# Autodesk Inventor assembly: test-model-2025dcm
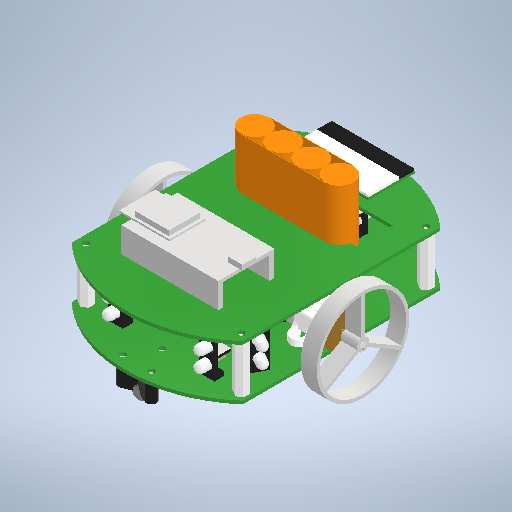
[picture p0: Inventor's stored thumbnail of the model, 512x512]
Saved by Autodesk Inventor 2025.3 (Build 293356000, 356)
## iProperties
Created: 2025-05-29
Part Number: test-model-2025dcm
Document SubType Name: Assembly
Designer: yamashita1
Author: yamashita1
## Documents named in this file (11)
- G:\マイドライブ\project\micro-mouse\3D-Model\test-model-2025dcm.iam
- G:\マイドライブ\project\micro-mouse\3D-Model\BaseBoard2.ipt
- G:\マイドライブ\project\micro-mouse\3D-Model\N20withBracket.iam
- G:\マイドライブ\project\micro-mouse\3D-Model\BallCaster-H16.ipt
- G:\マイドライブ\project\micro-mouse\3D-Model\D-Shaft_Wheel2.ipt
- G:\マイドライブ\project\micro-mouse\3D-Model\Photo-Sensor.iam
- G:\マイドライブ\project\micro-mouse\3D-Model\Spacer-M3H24.ipt
- G:\マイドライブ\project\micro-mouse\3D-Model\ESP32-DevKitC.ipt
- G:\マイドライブ\project\micro-mouse\3D-Model\NiMH-Battery.ipt
- G:\マイドライブ\project\micro-mouse\3D-Model\BaseBoard2B.ipt
- G:\マイドライブ\project\micro-mouse\3D-Model\AQM1602Y.ipt
## Components (19 placed, 10 different names)
1. BaseBoard2:1 — メイト:7, メイト:8, メイト:9, メイト:10, メイト:11, メイト:12, メイト:13, メイト:14, メイト:15, メイト:18, メイト:19, メイト:20, メイト:21, メイト:22, メイト:23, メイト:24, メイト:25, メイト:26, メイト:27, メイト:28, メイト:29, メイト:30, メイト:36
2. N20withBracket:1 [sub-assembly] — メイト:13, メイト:14, メイト:15, メイト:17, フラッシュ:2
3. N20withBracket:2 [sub-assembly] — メイト:10, メイト:11, メイト:12, メイト:16, フラッシュ:1
4. BallCaster-H16:1 — メイト:7, メイト:8, メイト:9
5. D-Shaft_Wheel2:1 — メイト:16, フラッシュ:1
6. D-Shaft_Wheel2:2 — メイト:17, フラッシュ:2
7. Photo-Sensor:1 [sub-assembly] — メイト:18
8. Photo-Sensor:2 [sub-assembly] — メイト:19
9. Photo-Sensor:3 [sub-assembly] — メイト:20
10. Photo-Sensor:4 [sub-assembly] — メイト:21
11. Photo-Sensor:5 [sub-assembly] — メイト:22
12. Spacer-M3H24:1 — メイト:23, メイト:29
13. Spacer-M3H24:2 — メイト:24, メイト:30, メイト:31, メイト:32
14. Spacer-M3H24:3 — メイト:25, メイト:27, メイト:33
15. Spacer-M3H24:4 — メイト:26, メイト:28
16. ESP32-DevKitC:1 — メイト:35
17. BaseBoard2B:1 — メイト:31, メイト:32, メイト:33, メイト:35
18. NiMH-Battery:1 — メイト:36
19. AQM1602Y:1
## Relationships (31: Mate 29, Flush 2)
- メイト:7 [Mate]: BaseBoard2:1 ↔ BallCaster-H16:1
- メイト:8 [Mate]: BaseBoard2:1 ↔ BallCaster-H16:1
- メイト:9 [Mate]: BaseBoard2:1 ↔ BallCaster-H16:1
- メイト:10 [Mate]: BaseBoard2:1 ↔ N20withBracket:2
- メイト:11 [Mate]: BaseBoard2:1 ↔ N20withBracket:2
- メイト:12 [Mate]: BaseBoard2:1 ↔ N20withBracket:2
- メイト:13 [Mate]: BaseBoard2:1 ↔ N20withBracket:1
- メイト:14 [Mate]: BaseBoard2:1 ↔ N20withBracket:1
- メイト:15 [Mate]: BaseBoard2:1 ↔ N20withBracket:1
- メイト:16 [Mate]: N20withBracket:2 ↔ D-Shaft_Wheel2:1
- フラッシュ:1 [Flush]: N20withBracket:2 ↔ D-Shaft_Wheel2:1
- メイト:17 [Mate]: N20withBracket:1 ↔ D-Shaft_Wheel2:2
- フラッシュ:2 [Flush]: N20withBracket:1 ↔ D-Shaft_Wheel2:2
- メイト:18 [Mate]: BaseBoard2:1 ↔ Photo-Sensor:1
- メイト:19 [Mate]: BaseBoard2:1 ↔ Photo-Sensor:2
- メイト:20 [Mate]: BaseBoard2:1 ↔ Photo-Sensor:3
- メイト:21 [Mate]: BaseBoard2:1 ↔ Photo-Sensor:4
- メイト:22 [Mate]: BaseBoard2:1 ↔ Photo-Sensor:5
- メイト:23 [Mate]: BaseBoard2:1 ↔ Spacer-M3H24:1
- メイト:24 [Mate]: BaseBoard2:1 ↔ Spacer-M3H24:2
- メイト:25 [Mate]: BaseBoard2:1 ↔ Spacer-M3H24:3
- メイト:26 [Mate]: BaseBoard2:1 ↔ Spacer-M3H24:4
- メイト:27 [Mate]: BaseBoard2:1 ↔ Spacer-M3H24:3
- メイト:28 [Mate]: BaseBoard2:1 ↔ Spacer-M3H24:4
- メイト:29 [Mate]: BaseBoard2:1 ↔ Spacer-M3H24:1
- メイト:30 [Mate]: BaseBoard2:1 ↔ Spacer-M3H24:2
- メイト:31 [Mate]: Spacer-M3H24:2 ↔ BaseBoard2B:1
- メイト:32 [Mate]: Spacer-M3H24:2 ↔ BaseBoard2B:1
- メイト:33 [Mate]: Spacer-M3H24:3 ↔ BaseBoard2B:1
- メイト:35 [Mate]: ESP32-DevKitC:1 ↔ BaseBoard2B:1
- メイト:36 [Mate]: BaseBoard2:1 ↔ NiMH-Battery:1
